# Autodesk Inventor assembly: NewGearboxAssembly
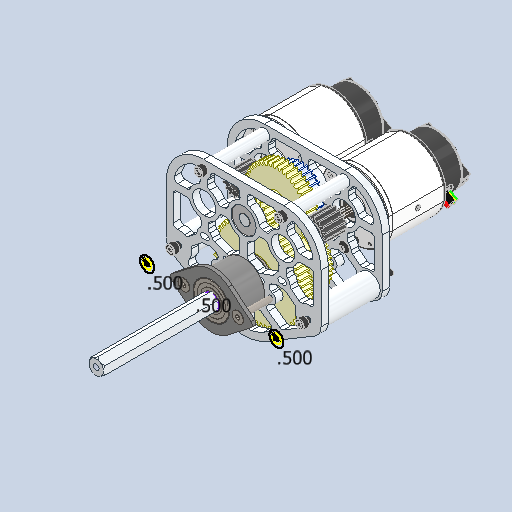
[picture p0: Inventor's stored thumbnail of the model, 512x512]
Saved by Autodesk Inventor 2022 (Build 260153000, 153)
## iProperties
Created: 2022-01-12
Part Number: NewGearboxAssembly
Document SubType Name: Assembly
Designer: merky
Author: merky
## Documents named in this file (6)
- C:\Users\tagaz\OneDrive\Documents\T3-Cad\CAD\2022 Parts\Generic\NewGearboxAssembly.iam
- C:\Users\tagaz\OneDrive\Documents\T3-Cad\CAD\2022 Parts\Generic\NewGearbox.ipt
- C:\Users\tagaz\OneDrive\Documents\T3-Cad\CAD\WCP DS Gearbox\217-3422-004 Rev2.ipt
- C:\Users\tagaz\OneDrive\Documents\T3-Cad\CAD\WCP DS Gearbox\217-3422-007 Rev1.ipt
- C:\Users\tagaz\OneDrive\Documents\T3-Cad\CAD\WCP DS Gearbox\217-2734.ipt
- C:\Users\tagaz\OneDrive\Documents\T3-Cad\CAD\2022 Parts\Generic\Falcon500.ipt
## Components (7 placed, 5 different names)
1. NewGearbox:1 — Insert:4, Insert:5, Insert:6
2. 217-3422-004 Rev2:1 — Insert:1, Insert:2, Insert:3
3. 217-3422-007 Rev1:1 — Insert:2
4. 217-3422-007 Rev1:2 — Insert:3
5. 217-2734:1 — Insert:1, Insert:4
6. Falcon500:1 — Insert:6
7. Falcon500:2 — Insert:5
## Relationships (6: Insert 6)
- Insert:1: 217-3422-004 Rev2:1 ↔ 217-2734:1
- Insert:2: 217-3422-004 Rev2:1 ↔ 217-3422-007 Rev1:1
- Insert:3: 217-3422-004 Rev2:1 ↔ 217-3422-007 Rev1:2
- Insert:4 (101.6 mm): NewGearbox:1 ↔ 217-2734:1
- Insert:5: NewGearbox:1 ↔ Falcon500:2
- Insert:6: NewGearbox:1 ↔ Falcon500:1
